# Autodesk Inventor assembly: Assembly29
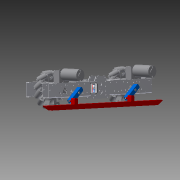
[picture p0: Inventor's stored thumbnail of the model, 180x180]
Saved by Autodesk Inventor 2014 (Build 180170000, 170)
## iProperties
Created: 2016-01-10
Part Number: Assembly29
Document SubType Name: Assembly
Designer: Applefamily
Author: Applefamily
## Documents named in this file (11)
- C:\Users\Applefamily\Documents\Inventor\Strong\Imported Components\Assembly29.iam
- C:\Users\Applefamily\Documents\Inventor\Strong\Imported Components\am-2951 AM14U2 Outside Sheet.ipt\am-2951 AM14U2 Outside Sheet.ipt.ipt
- C:\Users\Applefamily\Documents\Inventor\Strong\GearBox and Mec.iam
- C:\Users\Applefamily\Documents\Inventor\Strong\Imported Components\FR8ZZ Hex Bearing.ipt\FR8ZZ Hex Bearing.ipt.ipt
- C:\Users\Applefamily\Documents\Inventor\Strong\Imported Components\am-2952 AM14U2 Inside Sheet.ipt\am-2952 AM14U2 Inside Sheet.ipt.ipt
- C:\Users\Applefamily\Documents\Inventor\Strong\3inLink.ipt
- C:\Users\Applefamily\Documents\Inventor\Strong\Half Inch shaft.ipt
- C:\Users\Applefamily\Documents\Inventor\Strong\Skid.ipt
- am-2951 AM14U2 Outside Sheet.ipt
- FR8ZZ Hex Bearing.ipt
- am-2952 AM14U2 Inside Sheet.ipt
## Components (12 placed, 7 different names)
1. am-2951 AM14U2 Outside Sheet.ipt:1 — Cylindrical:1, Cylindrical:2, Mate:1, Mate:2
2. GearBox and Mec:1 [sub-assembly] — Cylindrical:4, Cylindrical:6, Flush:1, Mate:3, Rotational:2
3. FR8ZZ Hex Bearing.ipt:1 — Cylindrical:1, Mate:1, Cylindrical:6
4. FR8ZZ Hex Bearing.ipt:2 — Cylindrical:2, Mate:2, Cylindrical:3
5. GearBox and Mec:2 [sub-assembly] — Cylindrical:3, Cylindrical:5, Flush:1, Mate:4, Rotational:1
6. am-2952 AM14U2 Inside Sheet.ipt:1 — Cylindrical:4, Cylindrical:5, Mate:3, Mate:4
7. am-2952 AM14U2 Inside Sheet.ipt:2 — Rotational:1, Rotational:2, Flush:2, Cylindrical:7, Cylindrical:8, Mate:5, Mate:6
8. 3inLink:1 — Cylindrical:9, Mate:5, Cylindrical:11
9. Half Inch shaft:1 — Cylindrical:7, Cylindrical:9
10. Half Inch shaft:2 — Cylindrical:8, Cylindrical:10
11. 3inLink:2 — Cylindrical:10, Mate:6, Cylindrical:12, Mate:7
12. Skid:1 — Cylindrical:12, Cylindrical:11, Mate:7
## Relationships (23: CylindricalJoint 12, Mate 7, Flush 2, RevoluteJoint 2)
- Cylindrical:1: am-2951 AM14U2 Outside Sheet.ipt:1 ↔ FR8ZZ Hex Bearing.ipt:1
- Cylindrical:2: am-2951 AM14U2 Outside Sheet.ipt:1 ↔ FR8ZZ Hex Bearing.ipt:2
- Mate:1: am-2951 AM14U2 Outside Sheet.ipt:1 ↔ FR8ZZ Hex Bearing.ipt:1
- Mate:2: am-2951 AM14U2 Outside Sheet.ipt:1 ↔ FR8ZZ Hex Bearing.ipt:2
- Cylindrical:3: FR8ZZ Hex Bearing.ipt:2 ↔ GearBox and Mec:2
- Cylindrical:4: GearBox and Mec:1 ↔ am-2952 AM14U2 Inside Sheet.ipt:1
- Cylindrical:5: GearBox and Mec:2 ↔ am-2952 AM14U2 Inside Sheet.ipt:1
- Cylindrical:6: GearBox and Mec:1 ↔ FR8ZZ Hex Bearing.ipt:1
- Flush:1: GearBox and Mec:1 ↔ GearBox and Mec:2
- Mate:3: GearBox and Mec:1 ↔ am-2952 AM14U2 Inside Sheet.ipt:1
- Mate:4: GearBox and Mec:2 ↔ am-2952 AM14U2 Inside Sheet.ipt:1
- Rotational:1 [RevoluteJoint]: GearBox and Mec:2 ↔ am-2952 AM14U2 Inside Sheet.ipt:2
- Rotational:2 [RevoluteJoint]: GearBox and Mec:1 ↔ am-2952 AM14U2 Inside Sheet.ipt:2
- Flush:2 (25.4 mm): am-2952 AM14U2 Inside Sheet.ipt:2
- Cylindrical:7: am-2952 AM14U2 Inside Sheet.ipt:2 ↔ Half Inch shaft:1
- Cylindrical:8: am-2952 AM14U2 Inside Sheet.ipt:2 ↔ Half Inch shaft:2
- Cylindrical:9: 3inLink:1 ↔ Half Inch shaft:1
- Mate:5 (19.05 mm): am-2952 AM14U2 Inside Sheet.ipt:2 ↔ 3inLink:1
- Cylindrical:10: Half Inch shaft:2 ↔ 3inLink:2
- Mate:6 (19.05 mm): am-2952 AM14U2 Inside Sheet.ipt:2 ↔ 3inLink:2
- Cylindrical:12: 3inLink:2 ↔ Skid:1
- Cylindrical:11: 3inLink:1 ↔ Skid:1
- Mate:7: 3inLink:2 ↔ Skid:1
